# Autodesk Inventor assembly: Bumper Assembly
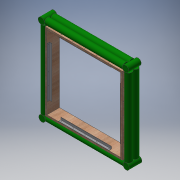
[picture p0: Inventor's stored thumbnail of the model, 180x180]
Saved by Autodesk Inventor 2018 (Build 220112000, 112)
## iProperties
Created: 2019-02-24
Part Number: Bumper Assembly
Document SubType Name: Assembly
Designer: maste
Author: maste
## Documents named in this file (3)
- C:\Users\s-2512711\Desktop\Github\2019CAD\Drivebase but Calvin is a mad man\Bumper Assembly.iam
- C:\Users\s-2512711\Desktop\Github\2019CAD\Drivebase but Calvin is a mad man\Bumper Side.ipt
- C:\Users\s-2512711\Desktop\Github\2019CAD\Drivebase but Calvin is a mad man\Bumper L.ipt
## Components (8 placed, 2 different names)
1. Bumper Side:1 — Mate:1, Flush:1, Flush:2, Mate:23, Mate:24, Mate:25
2. Bumper Side:2 — Mate:1, Flush:1, Flush:2, Flush:3, Flush:4, Mate:2, Mate:20, Mate:21, Mate:22
3. Bumper Side:3 — Flush:3, Flush:4, Mate:2, Flush:5, Flush:6, Mate:3, Mate:17, Mate:18, Mate:19
4. Bumper Side:4 — Flush:5, Flush:6, Mate:3, Mate:26, Mate:27, Mate:28
5. Bumper L:1 — Mate:26, Mate:27, Mate:28
6. Bumper L:2 — Mate:17, Mate:18, Mate:19
7. Bumper L:3 — Mate:20, Mate:21, Mate:22
8. Bumper L:4 — Mate:23, Mate:24, Mate:25
## Relationships (21: Mate 15, Flush 6)
- Mate:1: Bumper Side:1 ↔ Bumper Side:2
- Flush:1: Bumper Side:1 ↔ Bumper Side:2
- Flush:2: Bumper Side:1 ↔ Bumper Side:2
- Flush:3: Bumper Side:2 ↔ Bumper Side:3
- Flush:4: Bumper Side:2 ↔ Bumper Side:3
- Mate:2: Bumper Side:2 ↔ Bumper Side:3
- Flush:5: Bumper Side:3 ↔ Bumper Side:4
- Flush:6: Bumper Side:3 ↔ Bumper Side:4
- Mate:3: Bumper Side:3 ↔ Bumper Side:4
- Mate:17: Bumper Side:3 ↔ Bumper L:2
- Mate:18: Bumper Side:3 ↔ Bumper L:2
- Mate:19: Bumper Side:3 ↔ Bumper L:2
- Mate:20: Bumper Side:2 ↔ Bumper L:3
- Mate:21: Bumper Side:2 ↔ Bumper L:3
- Mate:22: Bumper Side:2 ↔ Bumper L:3
- Mate:23: Bumper Side:1 ↔ Bumper L:4
- Mate:24: Bumper Side:1 ↔ Bumper L:4
- Mate:25: Bumper Side:1 ↔ Bumper L:4
- Mate:26: Bumper Side:4 ↔ Bumper L:1
- Mate:27: Bumper Side:4 ↔ Bumper L:1
- Mate:28: Bumper Side:4 ↔ Bumper L:1
